# Autodesk Inventor assembly: Frame Layer open
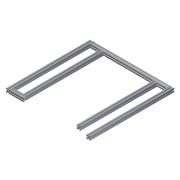
[picture p0: Inventor's stored thumbnail of the model, 180x180]
Saved by Autodesk Inventor 2013 (Build 170138000, 138)
## iProperties
Created: 2013-09-22
Part Number: Frame Layer open
Document SubType Name: Assembly
Designer: Family Room
Mass: 374.109 g
Surface Area: 4101.46 cm^2
Volume: 374.109 cm^3
Density: 1 g/cm^3
Author: Family Room
## Documents named in this file (4)
- C:\Users\kahohbein\Documents\GitHub\2013-2014_BlockParty\CAD\Drive\Final Drive Complete\Frame Layer open.iam
- C:\Users\kahohbein\Documents\GitHub\2013-2014_BlockParty\CAD\Drive\Final Drive Complete\Frame side.ipt
- C:\Users\kahohbein\Documents\GitHub\2013-2014_BlockParty\CAD\Drive\Final Drive Complete\Frontorback.ipt
- C:\Users\kahohbein\Documents\GitHub\2013-2014_BlockParty\CAD\Drive\Final Drive Complete\Inner side.ipt
## Components (5 placed, 3 different names)
1. Frame side:1 — Flush:11, Flush:12, Mate:9, Mate:13
2. Frame side:2 — Mate:1, Flush:1, Flush:2, Mate:11
3. Frontorback:1 — Mate:1, Flush:1, Flush:2, Flush:11, Flush:12, Mate:9, Mate:10, Flush:13, Mate:12, Flush:14
4. Inner side:1 — Mate:10, Flush:13, Mate:11
5. Inner side:2 — Mate:12, Flush:14, Mate:13
## Relationships (12: Mate 6, Flush 6)
- Mate:1: Frame side:2 ↔ Frontorback:1
- Flush:1: Frame side:2 ↔ Frontorback:1
- Flush:2: Frame side:2 ↔ Frontorback:1
- Flush:11: Frame side:1 ↔ Frontorback:1
- Flush:12: Frame side:1 ↔ Frontorback:1
- Mate:9: Frame side:1 ↔ Frontorback:1
- Mate:10: Frontorback:1 ↔ Inner side:1
- Flush:13: Frontorback:1 ↔ Inner side:1
- Mate:11 (50.8 mm): Frame side:2 ↔ Inner side:1
- Mate:12: Frontorback:1 ↔ Inner side:2
- Flush:14: Frontorback:1 ↔ Inner side:2
- Mate:13 (50.8 mm): Frame side:1 ↔ Inner side:2
